# Autodesk Inventor assembly: Spine
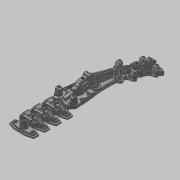
[picture p0: Inventor's stored thumbnail of the model, 180x180]
Saved by Autodesk Inventor 2015 SP1 (Build 190203100, 203)
## iProperties
Created: 2016-10-02
Part Number: Spine
Document SubType Name: Assembly
Designer: Val
Author: Val
## Documents named in this file (14)
- C:\Users\Val\Desktop\ExoGit\elysium-max-exoskeleton\src\Assemblies\Spine.iam
- C:\Users\Val\Desktop\ExoGit\elysium-max-exoskeleton\src\SpineBottom.ipt
- C:\Users\Val\Desktop\ExoGit\elysium-max-exoskeleton\src\SpineConnector.ipt
- C:\Users\Val\Desktop\ExoGit\elysium-max-exoskeleton\src\SpineCoverLeft.ipt
- C:\Users\Val\Desktop\ExoGit\elysium-max-exoskeleton\src\SpineCoverMiddle.ipt
- C:\Users\Val\Desktop\ExoGit\elysium-max-exoskeleton\src\SpineCoverRight.ipt
- C:\Users\Val\Desktop\ExoGit\elysium-max-exoskeleton\src\SpineLink.ipt
- C:\Users\Val\Desktop\ExoGit\elysium-max-exoskeleton\src\SpineMiddleLeft.ipt
- C:\Users\Val\Desktop\ExoGit\elysium-max-exoskeleton\src\SpineMiddleRight.ipt
- C:\Users\Val\Desktop\ExoGit\elysium-max-exoskeleton\src\SpineMiddleTop.ipt
- C:\Users\Val\Desktop\ExoGit\elysium-max-exoskeleton\src\SpineNeckLinkConnector.ipt
- C:\Users\Val\Desktop\ExoGit\elysium-max-exoskeleton\src\SpineTop.ipt
- C:\Users\Val\Desktop\ExoGit\elysium-max-exoskeleton\src\SpineTopMiddleConnector.ipt
- C:\Users\Val\Desktop\ExoGit\elysium-max-exoskeleton\src\SpacerLong.ipt
## Components (24 placed, 13 different names)
1. SpineBottom:1 — Mate:1, Mate:6, Mate:7, Mate:8, Mate:26, Mate:27, Mate:28, Mate:29, Mate:30, Angle:2, Mate:39, Mate:40, Mate:41, Mate:42
2. SpineConnector:1 — Mate:30, Angle:2, Mate:31, Angle:3, Flush:1
3. SpineCoverLeft:1 — Mate:26, Mate:27
4. SpineCoverMiddle:1 — Mate:2, Mate:3, Mate:4, Mate:5, Mate:8
5. SpineCoverRight:1 — Mate:28, Mate:29
6. SpineLink:1 — Mate:31, Angle:3, Mate:35
7. SpineMiddleLeft:1 — Mate:4, Mate:5, Mate:6, Mate:9, Mate:10, Angle:1, Mate:24
8. SpineMiddleRight:1 — Mate:2, Mate:3, Mate:7, Mate:9, Mate:11, Mate:12, Mate:19, Mate:20
9. SpineMiddleTop:1 — Mate:13, Mate:14, Mate:15, Mate:16, Angle:1, Mate:22, Mate:23
10. SpineNeckLinkConnector:1 — Mate:10, Mate:11, Mate:12, Mate:13, Mate:14, Mate:21
11. SpineTop:1 — Mate:15, Mate:16, Mate:43, Mate:44, Mate:45, Mate:46
12. SpineTopMiddleConnector:2 — Mate:19, Mate:20, Mate:21
13. SpineTopMiddleConnector:3 — Mate:22, Mate:23, Mate:24
14. SpineConnector:2 — Mate:35, Mate:36, Flush:1, Flush:2
15. SpineLink:2 — Angle:5, Mate:36, Mate:37
16. SpineConnector:3 — Mate:37, Flush:2, Mate:38, Flush:3
17. SpineLink:3 — Angle:5, Mate:38, Mate:47
18. SpacerLong:1 — Mate:41, Mate:42
19. SpacerLong:2 — Mate:39, Mate:40
20. SpacerLong:3 — Angle:6
21. SpacerLong:4 — Angle:6
22. SpacerLong:5 — Mate:45, Mate:46
23. SpacerLong:6 — Mate:43, Mate:44
24. SpineConnector:4 — Mate:47, Flush:3
## Relationships (50: Mate 41, Angle 6, Flush 3)
- Mate:1: SpineBottom:1
- Mate:2: SpineCoverMiddle:1 ↔ SpineMiddleRight:1
- Mate:3: SpineCoverMiddle:1 ↔ SpineMiddleRight:1
- Mate:4: SpineCoverMiddle:1 ↔ SpineMiddleLeft:1
- Mate:5: SpineCoverMiddle:1 ↔ SpineMiddleLeft:1
- Mate:6: SpineBottom:1 ↔ SpineMiddleLeft:1
- Mate:7: SpineBottom:1 ↔ SpineMiddleRight:1
- Mate:8: SpineBottom:1 ↔ SpineCoverMiddle:1
- Mate:9: SpineMiddleLeft:1 ↔ SpineMiddleRight:1
- Mate:10: SpineMiddleLeft:1 ↔ SpineNeckLinkConnector:1
- Mate:11: SpineMiddleRight:1 ↔ SpineNeckLinkConnector:1
- Mate:12: SpineMiddleRight:1 ↔ SpineNeckLinkConnector:1
- Mate:13: SpineMiddleTop:1 ↔ SpineNeckLinkConnector:1
- Mate:14: SpineMiddleTop:1 ↔ SpineNeckLinkConnector:1
- Mate:15: SpineMiddleTop:1 ↔ SpineTop:1
- Mate:16: SpineMiddleTop:1 ↔ SpineTop:1
- Angle:1 (180 deg): SpineMiddleLeft:1 ↔ SpineMiddleTop:1
- Mate:19: SpineMiddleRight:1 ↔ SpineTopMiddleConnector:2
- Mate:20: SpineMiddleRight:1 ↔ SpineTopMiddleConnector:2
- Mate:21: SpineNeckLinkConnector:1 ↔ SpineTopMiddleConnector:2
- Mate:22: SpineMiddleTop:1 ↔ SpineTopMiddleConnector:3
- Mate:23: SpineMiddleTop:1 ↔ SpineTopMiddleConnector:3
- Mate:24: SpineMiddleLeft:1 ↔ SpineTopMiddleConnector:3
- Mate:26: SpineBottom:1 ↔ SpineCoverLeft:1
- Mate:27: SpineBottom:1 ↔ SpineCoverLeft:1
- Mate:28: SpineBottom:1 ↔ SpineCoverRight:1
- Mate:29: SpineBottom:1 ↔ SpineCoverRight:1
- Mate:30: SpineBottom:1 ↔ SpineConnector:1
- Angle:2 (0 deg): SpineBottom:1 ↔ SpineConnector:1
- Mate:31: SpineConnector:1 ↔ SpineLink:1
- Angle:3 (0 deg): SpineConnector:1 ↔ SpineLink:1
- [Angle] (0 deg): SpineConnector:2 ↔ SpineLink:2
- Angle:5 (0 deg): SpineLink:2 ↔ SpineLink:3
- Mate:35: SpineLink:1 ↔ SpineConnector:2
- Mate:36: SpineConnector:2 ↔ SpineLink:2
- Mate:37: SpineLink:2 ↔ SpineConnector:3
- Flush:1: SpineConnector:1 ↔ SpineConnector:2
- Flush:2: SpineConnector:2 ↔ SpineConnector:3
- Mate:38: SpineConnector:3 ↔ SpineLink:3
- Mate:39: SpineBottom:1 ↔ SpacerLong:2
- Mate:40: SpineBottom:1 ↔ SpacerLong:2
- Mate:41: SpineBottom:1 ↔ SpacerLong:1
- Mate:42: SpineBottom:1 ↔ SpacerLong:1
- Mate:43: SpineTop:1 ↔ SpacerLong:6
- Mate:44: SpineTop:1 ↔ SpacerLong:6
- Mate:45: SpineTop:1 ↔ SpacerLong:5
- Mate:46: SpineTop:1 ↔ SpacerLong:5
- Angle:6 (0 deg): SpacerLong:3 ↔ SpacerLong:4
- Mate:47: SpineLink:3 ↔ SpineConnector:4
- Flush:3: SpineConnector:3 ↔ SpineConnector:4
## Named parameters: d37_d35 = 0 deg
